# Autodesk Inventor assembly: PCB
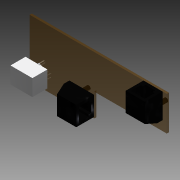
[picture p0: Inventor's stored thumbnail of the model, 180x180]
Saved by Autodesk Inventor 2014 (Build 180170000, 170)
## iProperties
Created: 2014-04-06
Part Number: PCB
Document SubType Name: Assembly
Designer: Tyler
Author: Tyler
## Documents named in this file (4)
- C:\Users\Tyler\Documents\ft8900cad\PCB\PCB.iam
- C:\Users\Tyler\Documents\ft8900cad\PCB\pcb.ipt
- C:\Users\Tyler\Documents\ft8900cad\PCB\USB_B.ipt
- C:\Users\Tyler\Documents\ft8900cad\PCB\6P6C.ipt
## Components (4 placed, 3 different names)
1. pcb:1 — Flush:1, Mate:1, Flush:2, Mate:2, Flush:3, Flush:4, Mate:3, Flush:5, Flush:6
2. USB_B:1 — Flush:1, Mate:1, Flush:2
3. 6P6C:1 — Mate:2, Flush:3, Flush:4
4. 6P6C:2 — Mate:3, Flush:5, Flush:6
## Relationships (9: Flush 6, Mate 3)
- Flush:1 (2 mm): pcb:1 ↔ USB_B:1
- Mate:1: pcb:1 ↔ USB_B:1
- Flush:2 (-3 mm): pcb:1 ↔ USB_B:1
- Mate:2: pcb:1 ↔ 6P6C:1
- Flush:3: pcb:1 ↔ 6P6C:1
- Flush:4 (1 mm): pcb:1 ↔ 6P6C:1
- Mate:3: pcb:1 ↔ 6P6C:2
- Flush:5: pcb:1 ↔ 6P6C:2
- Flush:6 (3 mm): pcb:1 ↔ 6P6C:2
